# Autodesk Inventor assembly: section_middle
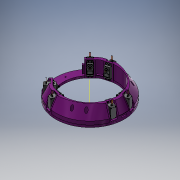
[picture p0: Inventor's stored thumbnail of the model, 180x180]
Saved by Autodesk Inventor 2017 (Build 210142000, 142)
## iProperties
Part Number: section_middle
Material: Ogólny
Document SubType Name: Assembly
Designer: Speed King
Mass: 489.559 g
Surface Area: 1645.04 cm^2
Volume: 481.359 cm^3
Density: 1.01703 g/cm^3
Author: Speed King
## Documents named in this file (7)
- C:\Users\Speed King\Documents\My Inventor\GrabCAD\Technical Informatics\CAD\model\section_ground.iam
- C:\Users\Speed King\Documents\My Inventor\GrabCAD\Technical Informatics\CAD\model\plate_ground.ipt
- C:\Users\Speed King\Documents\My Inventor\GrabCAD\Technical Informatics\CAD\model\Tower Pro MG955\TOWER PRO MG-995, ANALOG SERVO.iam
- C:\Users\Speed King\Documents\My Inventor\GrabCAD\Technical Informatics\CAD\model\bolts\Design Accelerator\section_ground_servo_upper.iam
- C:\Users\Speed King\Documents\My Inventor\GrabCAD\Technical Informatics\CAD\model\bolts\Design Accelerator\section_ground_servo_lower.iam
- C:\Users\Speed King\Documents\My Inventor\GrabCAD\Technical Informatics\CAD\model\connector.ipt
- C:\Users\Speed King\Documents\My Inventor\GrabCAD\Technical Informatics\CAD\model\connector_temp.ipt
## Components (22 placed, 5 different names)
1. plate_ground:1 — Zestawiający:1, Zestawiający:2, Zestawiający:3, Zestawiający:4, Zestawiający:5, Zestawiający:6, Zestawiający:7, Zestawiający:8, Zestawiający:9, Zestawiający:10, Zestawiający:11, Zestawiający:12, Równoległy:1, Zestawiający:13, Kąt:9, Kąt:7, Kąt:8, Kąt:10, Kąt:11, Kąt:12, Zestawiający:16, Zestawiający:18, Zestawiający:19, Zestawiający:20, Równoległy:2, Równoległy:3, Zestawiający:27, Zestawiający:28, Zestawiający:29, Zestawiający:30, Równoległy:4, Równoległy:5
2. TOWER PRO MG-995, ANALOG SERVO:1 [sub-assembly] — Zestawiający:5, Zestawiający:6, Kąt:9
3. TOWER PRO MG-995, ANALOG SERVO:2 [sub-assembly] — Zestawiający:1, Zestawiający:2, Zestawiający:14, Kąt:7
4. TOWER PRO MG-995, ANALOG SERVO:3 [sub-assembly] — Zestawiający:3, Zestawiający:4, Kąt:8, Zestawiający:15, Zestawiający:17
5. TOWER PRO MG-995, ANALOG SERVO:4 [sub-assembly] — Zestawiający:11, Zestawiający:12, Kąt:10
6. TOWER PRO MG-995, ANALOG SERVO:5 [sub-assembly] — Zestawiający:9, Zestawiający:10, Kąt:11
7. TOWER PRO MG-995, ANALOG SERVO:6 [sub-assembly] — Zestawiający:7, Zestawiający:8, Kąt:12
8. connector:1 — Równoległy:2, Równoległy:3, Zestawiający:27
9. connector:2 — Zestawiający:28, Zestawiający:29, Zestawiający:30
10. connector_temp:1 — Równoległy:4, Równoległy:5
11. Połączenie gwintowe:1 [sub-assembly] — Zestawiający:15, Zestawiający:16, Zestawiający:20
12. Połączenie gwintowe:2 [sub-assembly] — Zestawiający:17, Zestawiający:18, Zestawiający:19
13. Połączenie gwintowe:3 [sub-assembly]
14. Połączenie gwintowe:4 [sub-assembly]
15. Połączenie gwintowe:5 [sub-assembly]
16. Połączenie gwintowe:6 [sub-assembly]
17. Połączenie gwintowe:7 [sub-assembly]
18. Połączenie gwintowe:8 [sub-assembly]
19. Połączenie gwintowe:9 [sub-assembly]
20. Połączenie gwintowe:10 [sub-assembly]
21. Połączenie gwintowe:11 [sub-assembly]
22. Połączenie gwintowe:12 [sub-assembly]
## Component patterns: (3 elements), (2 elements, first: Połączenie gwintowe:1 + Połączenie gwintowe:2), Szyk komponentów 1:2 (2 elements), Szyk komponentów 1:3 (2 elements)
## Relationships (35: Mate 24, Angle 6, Flush 5)
- Zestawiający:1 [Mate]: plate_ground:1 ↔ TOWER PRO MG-995, ANALOG SERVO:2
- Zestawiający:2 [Mate]: plate_ground:1 ↔ TOWER PRO MG-995, ANALOG SERVO:2
- Zestawiający:3 [Mate]: plate_ground:1 ↔ TOWER PRO MG-995, ANALOG SERVO:3
- Zestawiający:4 [Mate]: plate_ground:1 ↔ TOWER PRO MG-995, ANALOG SERVO:3
- Zestawiający:5 [Mate]: plate_ground:1 ↔ TOWER PRO MG-995, ANALOG SERVO:1
- Zestawiający:6 [Mate]: plate_ground:1 ↔ TOWER PRO MG-995, ANALOG SERVO:1
- Zestawiający:7 [Mate]: plate_ground:1 ↔ TOWER PRO MG-995, ANALOG SERVO:6
- Zestawiający:8 [Mate]: plate_ground:1 ↔ TOWER PRO MG-995, ANALOG SERVO:6
- Zestawiający:9 [Mate]: plate_ground:1 ↔ TOWER PRO MG-995, ANALOG SERVO:5
- Zestawiający:10 [Mate]: plate_ground:1 ↔ TOWER PRO MG-995, ANALOG SERVO:5
- Zestawiający:11 [Mate]: plate_ground:1 ↔ TOWER PRO MG-995, ANALOG SERVO:4
- Zestawiający:12 [Mate]: plate_ground:1 ↔ TOWER PRO MG-995, ANALOG SERVO:4
- Równoległy:1 [Flush]: plate_ground:1
- Zestawiający:13 [Mate]: plate_ground:1
- Zestawiający:14 [Mate]: TOWER PRO MG-995, ANALOG SERVO:2
- Kąt:9 [Angle] (0 deg): plate_ground:1 ↔ TOWER PRO MG-995, ANALOG SERVO:1
- Kąt:7 [Angle] (0 deg): plate_ground:1 ↔ TOWER PRO MG-995, ANALOG SERVO:2
- Kąt:8 [Angle] (0 deg): plate_ground:1 ↔ TOWER PRO MG-995, ANALOG SERVO:3
- Kąt:10 [Angle] (0 deg): plate_ground:1 ↔ TOWER PRO MG-995, ANALOG SERVO:4
- Kąt:11 [Angle] (0 deg): plate_ground:1 ↔ TOWER PRO MG-995, ANALOG SERVO:5
- Kąt:12 [Angle] (0 deg): plate_ground:1 ↔ TOWER PRO MG-995, ANALOG SERVO:6
- Zestawiający:15 [Mate]: TOWER PRO MG-995, ANALOG SERVO:3 ↔ Połączenie gwintowe:1
- Zestawiający:16 [Mate]: plate_ground:1 ↔ Połączenie gwintowe:1
- Zestawiający:17 [Mate]: TOWER PRO MG-995, ANALOG SERVO:3 ↔ Połączenie gwintowe:2
- Zestawiający:18 [Mate]: plate_ground:1 ↔ Połączenie gwintowe:2
- Zestawiający:19 [Mate]: plate_ground:1 ↔ Połączenie gwintowe:2
- Zestawiający:20 [Mate]: plate_ground:1 ↔ Połączenie gwintowe:1
- Równoległy:2 [Flush]: plate_ground:1 ↔ connector:1
- Równoległy:3 [Flush]: plate_ground:1 ↔ connector:1
- Zestawiający:27 [Mate]: plate_ground:1 ↔ connector:1
- Zestawiający:28 [Mate] (0.2 mm): plate_ground:1 ↔ connector:2
- Zestawiający:29 [Mate]: plate_ground:1 ↔ connector:2
- Zestawiający:30 [Mate] (0.2 mm): plate_ground:1 ↔ connector:2
- Równoległy:4 [Flush]: plate_ground:1 ↔ connector_temp:1
- Równoległy:5 [Flush]: plate_ground:1 ↔ connector_temp:1
